# Autodesk Inventor assembly: NanoCase
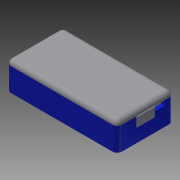
[picture p0: Inventor's stored thumbnail of the model, 180x180]
Saved by Autodesk Inventor 2014 SP1 (Build 180222100, 222)
## iProperties
Created: 2017-05-21
Part Number: NanoCase
Document SubType Name: Assembly
Designer: danielsikar
Author: danielsikar
## Documents named in this file (4)
- C:\Users\danielsikar\Documents\Inventor\FlaskCradle\assemblies\NanoCase.iam
- C:\Users\danielsikar\Documents\Inventor\FlaskCradle\parts\ArduinoNano.ipt
- C:\Users\danielsikar\Documents\Inventor\FlaskCradle\parts\NanoCaseBottom.ipt
- C:\Users\danielsikar\Documents\Inventor\FlaskCradle\parts\NanoCaseTop.ipt
## Components (3 placed, 3 different names)
1. ArduinoNano:1 — Mate:1, Mate:2, Mate:3, Flush:1
2. NanoCaseBottom:1 — Flush:2, Flush:3, Flush:4
3. NanoCaseTop:1 — Flush:3, Flush:4
## Relationships (7: Flush 4, Mate 3)
- Mate:1: ArduinoNano:1
- Mate:2: ArduinoNano:1
- Mate:3: ArduinoNano:1
- Flush:1 (2 mm): ArduinoNano:1
- Flush:2: NanoCaseBottom:1
- Flush:3: NanoCaseBottom:1 ↔ NanoCaseTop:1
- Flush:4: NanoCaseBottom:1 ↔ NanoCaseTop:1
